# Autodesk Inventor assembly: ParallelLinksDriveUnit_MIR
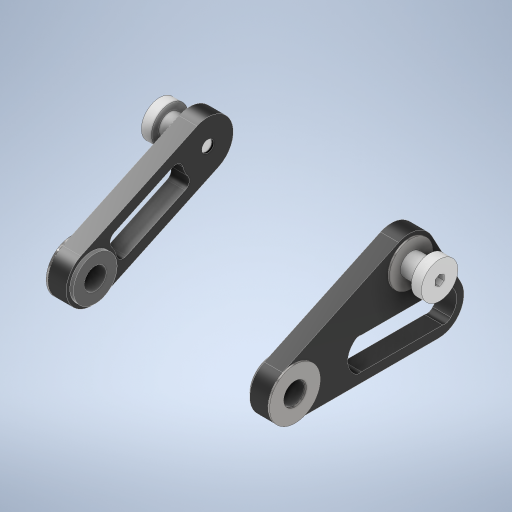
[picture p0: Inventor's stored thumbnail of the model, 512x512]
Saved by Autodesk Inventor 2024.2 (Build 282272000, 272)
## iProperties
Created: 2024-01-07
Part Number: ParallelLinksDriveUnit_MIR
Document SubType Name: Assembly
Designer: Masato Kubotera
Mass: 29.5079 g
Surface Area: 81.9927 cm^2
Volume: 9.0872 cm^3
Density: 3.24719 g/cm^3
Author: Masato Kubotera
## Documents named in this file (7)
- C:\Users\masato\OneDrive - Chiba Institute of Technology\CIT Brains\RoboCup2024\Mechanic\SUSTAINA-OP2\NativeFiles\Boby\LowerLimb\Legs\Links\ParallelLinksDriveUnit_MIR.iam
- C:\Users\masato\OneDrive - Chiba Institute of Technology\CIT Brains\RoboCup2024\Mechanic\SUSTAINA-OP2\NativeFiles\Boby\LowerLimb\Legs\Links\ParallelLinksDriveFrame.ipt
- C:\Users\masato\OneDrive - Chiba Institute of Technology\CIT Brains\RoboCup2024\Mechanic\SUSTAINA-OP2\NativeFiles\Boby\COTS\Bushes\GFM-0608-06.ipt
- C:\Users\masato\OneDrive - Chiba Institute of Technology\CIT Brains\RoboCup2024\Mechanic\SUSTAINA-OP2\NativeFiles\Boby\COTS\Washers\Metal\UUW-0614-05H.ipt
- C:\Users\masato\OneDrive - Chiba Institute of Technology\CIT Brains\RoboCup2024\Mechanic\SUSTAINA-OP2\NativeFiles\Boby\COTS\Washers\Metal\UUW-0412-05H.ipt
- C:\Users\masato\OneDrive - Chiba Institute of Technology\CIT Brains\RoboCup2024\Mechanic\SUSTAINA-OP2\NativeFiles\Boby\COTS\Screws\ScrewsWithShoulder\DBTSY4-5-5-DHC-PC.ipt
- C:\Users\masato\OneDrive - Chiba Institute of Technology\CIT Brains\RoboCup2024\Mechanic\SUSTAINA-OP2\NativeFiles\Boby\LowerLimb\Legs\Links\ParallelLinksDriveSimpleFrame.ipt
## Components (10 placed, 6 different names)
1. ParallelLinksDriveFrame:3 — Symmetry:1
2. ParallelLinksDriveSimpleFrame:1 — Symmetry:1, Insert:7, Insert:8, Insert:5
3. DBTSY4-5-5-DHC-PC:2 — Insert:4
4. DBTSY4-5-5-DHC-PC:1 — Insert:6
5. GFM-0608-06:1
6. GFM-0608-06:2 — Insert:8
7. UUW-0614-05H:1
8. UUW-0412-05H:1 — Insert:4
9. UUW-0614-05H:2 — Insert:7
10. UUW-0412-05H:2 — Insert:5, Insert:6
## Relationships (14: Insert 8, Flush 3, Mate 1, Angle 1, Symmetry 1)
- [Mate]: ParallelLinksDriveFrame:3
- [Angle] (0 deg): ParallelLinksDriveFrame:3
- [Flush] (25.25 mm): ParallelLinksDriveFrame:3
- [Insert]: ParallelLinksDriveFrame:3 ↔ GFM-0608-06:1
- [Insert]: ParallelLinksDriveFrame:3 ↔ UUW-0614-05H:1
- [Insert]: ParallelLinksDriveFrame:3 ↔ UUW-0412-05H:1
- Insert:4: DBTSY4-5-5-DHC-PC:2 ↔ UUW-0412-05H:1
- [Flush]: ParallelLinksDriveFrame:3 ↔ ParallelLinksDriveSimpleFrame:1
- [Flush]: ParallelLinksDriveFrame:3 ↔ ParallelLinksDriveSimpleFrame:1
- Symmetry:1: ParallelLinksDriveFrame:3 ↔ ParallelLinksDriveSimpleFrame:1
- Insert:5: ParallelLinksDriveSimpleFrame:1 ↔ UUW-0412-05H:2
- Insert:6: DBTSY4-5-5-DHC-PC:1 ↔ UUW-0412-05H:2
- Insert:7: ParallelLinksDriveSimpleFrame:1 ↔ UUW-0614-05H:2
- Insert:8: ParallelLinksDriveSimpleFrame:1 ↔ GFM-0608-06:2
